# Autodesk Inventor assembly: USB 3.0 A Recepticle
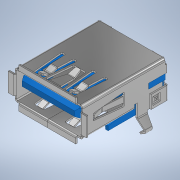
[picture p0: Inventor's stored thumbnail of the model, 180x180]
Saved by Autodesk Inventor 2020.1 (Build 241239000, 239)
## iProperties
Created: 2019-11-22
Part Number: USB 3.0 A Recepticle
Document SubType Name: Assembly
Designer: S. Lee
Mass: 2.37354 g
Surface Area: 30.7789 cm^2
Volume: 0.577297 cm^3
Density: 4.11146 g/cm^3
Author: S. Lee
## Documents named in this file (6)
- X:\AutoDesk\InventorProjects\Library\Electrical\Connectors\Comercial Connectors\USB\USB 3.0 A Recepticle.iam
- X:\AutoDesk\InventorProjects\Library\Electrical\Connectors\Comercial Connectors\USB\Parts\USB 3.0 A Recepticle Shell.ipt
- X:\AutoDesk\InventorProjects\Library\Electrical\Connectors\Comercial Connectors\USB\Parts\USB 3.0 A Recepticle Insert Fit.ipt
- X:\AutoDesk\InventorProjects\Library\Electrical\Connectors\Comercial Connectors\USB\Parts\USB 3.0 A Recepticle Upper Pin.ipt
- X:\AutoDesk\InventorProjects\Library\Electrical\Connectors\Comercial Connectors\USB\Parts\USB 3.0 A Recepticle Rear Insert Fit.ipt
- X:\AutoDesk\InventorProjects\Library\Electrical\Connectors\Comercial Connectors\USB\Parts\USB 3.0 A Recepticle Lower Pin.ipt
## Components (12 placed, 12 different names)
1. USB 3.0 A Recepticle Shell:1 — Mate:1, Flush:1, Mate:2
2. USB 3.0 A Recepticle Insert Fit:1 — Mate:1, Flush:1, Mate:2, Mate:3, Mate:4, Flush:2, Mate:6, Flush:3, Mate:7, Flush:4, Mate:8, Flush:5, Mate:9, Flush:6, Mate:10, Mate:11, Mate:12, Flush:7, Mate:13, Mate:14, Flush:8, Mate:15, Mate:16, Flush:9, Mate:17, Mate:18, Flush:10, Mate:19, Mate:20, Flush:11, Mate:21, Mate:22, Flush:12
3. USB 3.0 A Recepticle Rear Insert Fit:1 — Flush:2, Mate:6, Flush:3
4. Position 1 — Mate:7, Mate:8, Flush:5
5. Position 2 — Mate:17, Mate:18, Flush:10
6. Position 3 — Mate:19, Mate:20, Flush:11
7. Position 4 — Mate:21, Mate:22, Flush:12
8. Position 5 — Mate:3, Mate:4, Flush:4
9. Position 6 — Mate:9, Flush:6, Mate:10
10. Position 7 — Mate:11, Mate:12, Flush:7
11. Position 8 — Mate:13, Mate:14, Flush:8
12. Position 9 — Mate:15, Mate:16, Flush:9
## Relationships (33: Mate 21, Flush 12)
- Mate:1: USB 3.0 A Recepticle Shell:1 ↔ USB 3.0 A Recepticle Insert Fit:1
- Flush:1: USB 3.0 A Recepticle Shell:1 ↔ USB 3.0 A Recepticle Insert Fit:1
- Mate:2: USB 3.0 A Recepticle Shell:1 ↔ USB 3.0 A Recepticle Insert Fit:1
- Mate:3: USB 3.0 A Recepticle Insert Fit:1 ↔ Position 5
- Mate:4: USB 3.0 A Recepticle Insert Fit:1 ↔ Position 5
- Flush:2: USB 3.0 A Recepticle Insert Fit:1 ↔ USB 3.0 A Recepticle Rear Insert Fit:1
- Mate:6: USB 3.0 A Recepticle Insert Fit:1 ↔ USB 3.0 A Recepticle Rear Insert Fit:1
- Flush:3: USB 3.0 A Recepticle Insert Fit:1 ↔ USB 3.0 A Recepticle Rear Insert Fit:1
- Mate:7: USB 3.0 A Recepticle Insert Fit:1 ↔ Position 1
- Flush:4: USB 3.0 A Recepticle Insert Fit:1 ↔ Position 5
- Mate:8: USB 3.0 A Recepticle Insert Fit:1 ↔ Position 1
- Flush:5: USB 3.0 A Recepticle Insert Fit:1 ↔ Position 1
- Mate:9: USB 3.0 A Recepticle Insert Fit:1 ↔ Position 6
- Flush:6: USB 3.0 A Recepticle Insert Fit:1 ↔ Position 6
- Mate:10: USB 3.0 A Recepticle Insert Fit:1 ↔ Position 6
- Mate:11: USB 3.0 A Recepticle Insert Fit:1 ↔ Position 7
- Mate:12: USB 3.0 A Recepticle Insert Fit:1 ↔ Position 7
- Flush:7: USB 3.0 A Recepticle Insert Fit:1 ↔ Position 7
- Mate:13: USB 3.0 A Recepticle Insert Fit:1 ↔ Position 8
- Mate:14: USB 3.0 A Recepticle Insert Fit:1 ↔ Position 8
- Flush:8: USB 3.0 A Recepticle Insert Fit:1 ↔ Position 8
- Mate:15: USB 3.0 A Recepticle Insert Fit:1 ↔ Position 9
- Mate:16: USB 3.0 A Recepticle Insert Fit:1 ↔ Position 9
- Flush:9: USB 3.0 A Recepticle Insert Fit:1 ↔ Position 9
- Mate:17: USB 3.0 A Recepticle Insert Fit:1 ↔ Position 2
- Mate:18: USB 3.0 A Recepticle Insert Fit:1 ↔ Position 2
- Flush:10: USB 3.0 A Recepticle Insert Fit:1 ↔ Position 2
- Mate:19: USB 3.0 A Recepticle Insert Fit:1 ↔ Position 3
- Mate:20: USB 3.0 A Recepticle Insert Fit:1 ↔ Position 3
- Flush:11: USB 3.0 A Recepticle Insert Fit:1 ↔ Position 3
- Mate:21: USB 3.0 A Recepticle Insert Fit:1 ↔ Position 4
- Mate:22: USB 3.0 A Recepticle Insert Fit:1 ↔ Position 4
- Flush:12: USB 3.0 A Recepticle Insert Fit:1 ↔ Position 4
